# Autodesk Inventor assembly: switchback-exploded
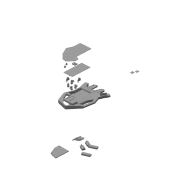
[picture p0: Inventor's stored thumbnail of the model, 180x180]
Saved by Autodesk Inventor 2020 (Build 240168000, 168)
## iProperties
Created: 2020-01-02
Part Number: switchback-exploded
Document SubType Name: Assembly
Designer: valer
Author: valer
## Documents named in this file (16)
- C:\Users\valer\Desktop\switchback\src\switchback-exploded.iam
- C:\Users\valer\Desktop\switchback\src\switchback.ipt
- C:\Users\valer\Desktop\switchback\src\strandberg-headless-tuner.ipt
- C:\Users\valer\Desktop\switchback\src\fishman-modern6.ipt
- C:\Users\valer\Desktop\switchback\src\fishman-modern8.ipt
- C:\Users\valer\Desktop\switchback\src\fishman-pot.ipt
- C:\Users\valer\Desktop\switchback\src\fishman-switch.ipt
- C:\Users\valer\Desktop\switchback\src\fishman-battery.ipt
- C:\Users\valer\Desktop\switchback\src\fishman-jack.ipt
- C:\Users\valer\Desktop\switchback\src\arduino.ipt
- C:\Users\valer\Desktop\switchback\src\oscilloscope-screen.ipt
- C:\Users\valer\Desktop\switchback\src\seaboard-block-keyboard.ipt
- C:\Users\valer\Desktop\switchback\src\seaboard-block-circuit-board.ipt
- C:\Users\valer\Desktop\switchback\src\switchback-electronics-cover.ipt
- C:\Users\valer\Desktop\switchback\src\switchback-logo.ipt
- C:\Users\valer\Desktop\switchback\src\switchback-logo-cover.ipt
## Components (35 placed, 15 different names)
1. switchback:1 — Mate:1, Mate:2, Mate:4, Mate:5, Mate:6, Mate:7, Mate:8, Mate:9, Mate:10, Mate:11, Mate:12, Mate:13, Mate:14, Mate:15, Mate:16, Mate:17, Mate:28, Mate:29, Mate:42, Mate:43, Mate:44, Mate:45, Mate:46, Mate:47, Mate:48, Mate:49, Mate:50, Mate:51, Mate:52, Mate:53, Mate:55, Mate:56, Mate:58, Mate:59, Mate:61, Mate:62, Mate:136, Mate:137, Mate:139, Mate:141, Mate:144, Mate:145, Mate:147, Mate:148, Mate:150, Mate:151, Mate:152, Mate:156, Mate:158, Mate:159, Mate:160, Mate:167, Mate:176, Mate:177, Mate:178, Mate:179
2. strandberg-headless-tuner:1 — Mate:1, Mate:2
3. strandberg-headless-tuner:2 — Mate:4, Mate:5
4. strandberg-headless-tuner:3 — Mate:6, Mate:7
5. strandberg-headless-tuner:4 — Mate:10, Mate:11
6. strandberg-headless-tuner:5 — Mate:12, Mate:13
7. strandberg-headless-tuner:6 — Mate:8, Mate:9
8. strandberg-headless-tuner:8 — Mate:14, Mate:15
9. strandberg-headless-tuner:9 — Mate:16, Mate:17
10. strandberg-headless-tuner:15 — Mate:28, Mate:29
11. strandberg-headless-tuner:16 — Mate:46, Mate:47
12. strandberg-headless-tuner:17 — Mate:48, Mate:49
13. strandberg-headless-tuner:18 — Mate:42, Mate:43
14. strandberg-headless-tuner:19 — Mate:44, Mate:45
15. strandberg-headless-tuner:20 — Mate:50, Mate:51
16. fishman-modern6:1 — Mate:52, Mate:53
17. fishman-modern6:2 — Mate:55, Mate:56
18. fishman-modern8:1 — Mate:61, Mate:62
19. fishman-modern8:2 — Mate:58, Mate:59
20. fishman-pot:4 — Mate:141
21. fishman-pot:5 — Mate:139
22. fishman-battery:1 — Mate:162, Angle:3
23. fishman-jack:1 — Mate:163
24. fishman-jack:2 — Mate:165
25. arduino:1 — Mate:155
26. OscilloscopeScreen:1 — Mate:150, Mate:151, Mate:152, Mate:155
27. seaboard-block-circuit-board:1 — Mate:167
28. fishman-switch:2 — Mate:147, Mate:148
29. seaboard-block-keyboard:1 — Mate:156
30. fishman-switch:3 — Mate:136, Mate:137
31. fishman-pot:6 — Mate:145
32. fishman-pot:7 — Mate:144
33. switchback-electronics-cover:1 — Mate:158, Mate:159, Mate:160, Mate:162, Angle:3, Mate:163, Mate:165
34. switchback-logo:1
35. switchback-logo-cover:1 — Mate:176, Mate:177, Mate:178, Mate:179
## Relationships (61: Mate 60, Angle 1)
- Mate:1: switchback:1 ↔ strandberg-headless-tuner:1
- Mate:2: switchback:1 ↔ strandberg-headless-tuner:1
- Mate:4: switchback:1 ↔ strandberg-headless-tuner:2
- Mate:5: switchback:1 ↔ strandberg-headless-tuner:2
- Mate:6: switchback:1 ↔ strandberg-headless-tuner:3
- Mate:7: switchback:1 ↔ strandberg-headless-tuner:3
- Mate:8: switchback:1 ↔ strandberg-headless-tuner:6
- Mate:9: switchback:1 ↔ strandberg-headless-tuner:6
- Mate:10: switchback:1 ↔ strandberg-headless-tuner:4
- Mate:11: switchback:1 ↔ strandberg-headless-tuner:4
- Mate:12: switchback:1 ↔ strandberg-headless-tuner:5
- Mate:13: switchback:1 ↔ strandberg-headless-tuner:5
- Mate:14: switchback:1 ↔ strandberg-headless-tuner:8
- Mate:15: switchback:1 ↔ strandberg-headless-tuner:8
- Mate:16: switchback:1 ↔ strandberg-headless-tuner:9
- Mate:17: switchback:1 ↔ strandberg-headless-tuner:9
- Mate:28: switchback:1 ↔ strandberg-headless-tuner:15
- Mate:29: switchback:1 ↔ strandberg-headless-tuner:15
- Mate:42: switchback:1 ↔ strandberg-headless-tuner:18
- Mate:43: switchback:1 ↔ strandberg-headless-tuner:18
- Mate:44: switchback:1 ↔ strandberg-headless-tuner:19
- Mate:45: switchback:1 ↔ strandberg-headless-tuner:19
- Mate:46: switchback:1 ↔ strandberg-headless-tuner:16
- Mate:47: switchback:1 ↔ strandberg-headless-tuner:16
- Mate:48: switchback:1 ↔ strandberg-headless-tuner:17
- Mate:49: switchback:1 ↔ strandberg-headless-tuner:17
- Mate:50: switchback:1 ↔ strandberg-headless-tuner:20
- Mate:51: switchback:1 ↔ strandberg-headless-tuner:20
- Mate:52: switchback:1 ↔ fishman-modern6:1
- Mate:53: switchback:1 ↔ fishman-modern6:1
- Mate:55: switchback:1 ↔ fishman-modern6:2
- Mate:56: switchback:1 ↔ fishman-modern6:2
- Mate:58: switchback:1 ↔ fishman-modern8:2
- Mate:59: switchback:1 ↔ fishman-modern8:2
- Mate:61: switchback:1 ↔ fishman-modern8:1
- Mate:62: switchback:1 ↔ fishman-modern8:1
- Mate:136: switchback:1 ↔ fishman-switch:3
- Mate:137: switchback:1 ↔ fishman-switch:3
- Mate:139: switchback:1 ↔ fishman-pot:5
- Mate:141: switchback:1 ↔ fishman-pot:4
- Mate:144: switchback:1 ↔ fishman-pot:7
- Mate:145: switchback:1 ↔ fishman-pot:6
- Mate:147: switchback:1 ↔ fishman-switch:2
- Mate:148: switchback:1 ↔ fishman-switch:2
- Mate:150: switchback:1 ↔ OscilloscopeScreen:1
- Mate:151: switchback:1 ↔ OscilloscopeScreen:1
- Mate:152: switchback:1 ↔ OscilloscopeScreen:1
- Mate:155: arduino:1 ↔ OscilloscopeScreen:1
- Mate:156: switchback:1 ↔ seaboard-block-keyboard:1
- Mate:158: switchback:1 ↔ switchback-electronics-cover:1
- Mate:159: switchback:1 ↔ switchback-electronics-cover:1
- Mate:160: switchback:1 ↔ switchback-electronics-cover:1
- Mate:162: fishman-battery:1 ↔ switchback-electronics-cover:1
- Angle:3 (0 deg): fishman-battery:1 ↔ switchback-electronics-cover:1
- Mate:163: fishman-jack:1 ↔ switchback-electronics-cover:1
- Mate:165: fishman-jack:2 ↔ switchback-electronics-cover:1
- Mate:167: switchback:1 ↔ seaboard-block-circuit-board:1
- Mate:176: switchback:1 ↔ switchback-logo-cover:1
- Mate:177: switchback:1 ↔ switchback-logo-cover:1
- Mate:178: switchback:1 ↔ switchback-logo-cover:1
- Mate:179: switchback:1 ↔ switchback-logo-cover:1
